# Autodesk Inventor assembly: Main
(part 2 of 2)
- Insert:313 (-2 mm): Extruder:1 ↔ 90729A168_Passivated 316 :6
- Insert:314 (-2 mm): Extruder:1 ↔ 90729A168_Passivated 316 :7
- Insert:315: ThrustBearing:4 ↔ ElevatorShoulderBoltMount:1
- Insert:316: ScissorArmV2Inner:1 ↔ ThrustBearing:4
- Insert:317: ScissorArmV2Inner_MIR:1 ↔ ThrustBearing:5
- Mate:181: ElevatorShoulderBoltMount_MIR:1 ↔ ThrustBearing:5
- Mate:182 (0.16 mm): Tensioner:1 ↔ RoutingPlateV2:1
- Mate:183 (0.16 mm): RoutingPlateV2Right:1 ↔ Tensioner:2
- Insert:318: ElevatorShoulderBoltMount:1 ↔ 91415A210_Zinc-Plated Steel Hex Nut:3
- Mate:184: ElevatorPlate_MIR:1 ↔ ElevatorShoulderBoltMount_MIR:1
- Insert:319: MGNRail250mm:4 ↔ GantryRailMount:1
- Insert:320: MGNRail250mm:4 ↔ GantryRailMount:1
- Insert:321: BearingU604:1 ↔ GantryRailMount:1
- Insert:322: ElevatorPlate:1 ↔ MGNRail250mm:10
- Insert:323: ElevatorPlate:1 ↔ MGNRail250mm:10
- Flush:51 (-5.5 mm): MGN9-C v2:1 ↔ MGNRail250mm:10
- Insert:324: 7804K117_Stainless Steel Ball Bearing_MIR:1 ↔ ScissorArmV2Inner_MIR:1
- Insert:325: 7804K117_Stainless Steel Ball Bearing:2 ↔ ScissorArmV2Inner:1
- Insert:326: ScissorArmV2Inner:1 ↔ 7804K117_Stainless Steel Ball Bearing:8
- Insert:327: ScissorArmV2Inner_MIR:1 ↔ 7804K117_Stainless Steel Ball Bearing_MIR:5
- Mate:185: MGN9-H:2 ↔ MGNRail250mm:8
- Flush:52: BottomSideMountRight:1 ↔ RightTruss:1
- Mate:186: ScissorArmV2Inner_MIR:1 ↔ 6656K108_Steel Ball Bearing_MIR:2
- Insert:328: BottomSlideMount:1 ↔ LeftLevelBlock:1
- Flush:53: BottomSlideMount:1 ↔ LeftLevelBlock:1
- Insert:329: BottomSideMountRight:1 ↔ RightLevelBlock:1
- Flush:54: BottomSideMountRight:1 ↔ RightLevelBlock:1
- Insert:330: BottomSlideMountExtension_MIR:1 ↔ FrontLevelBlock:1
- Mate:187: BottomSlideMountExtension_MIR:1 ↔ FrontLevelBlock:1
- Insert:331: FrontLevelBlock:1 ↔ Spring8x20mm:1
- Insert:332: RightLevelBlock:1 ↔ Spring8x20mm:3
- Insert:333: LeftLevelBlock:1 ↔ Spring8x20mm:2
- Mate:188: MGNRail250mm:7 ↔ ElevatorPlate_MIR:1
- Insert:334: ElevatorPlate:1 ↔ Nema17x38mm:1
- Mate:189: ElevatorPlate:1 ↔ Nema17x38mm:1
- Insert:335: ElevatorPlate_MIR:1 ↔ Nema17x38mm:2
- Mate:190: ElevatorPlate_MIR:1 ↔ Nema17x38mm:2
- Mate:191: Pulley:2 ↔ Nema17x38mm:2
- Mate:192: Pulley:1 ↔ Nema17x38mm:1
- Flush:55: Pulley:1 ↔ Pulley:2
## Named parameters: d361_d326 = 0 mm, d362_d327 = 5.5 mm, d552_d463 = 0 mm, d553_d540 = 0 mm
